# Autodesk Inventor assembly: PI-101
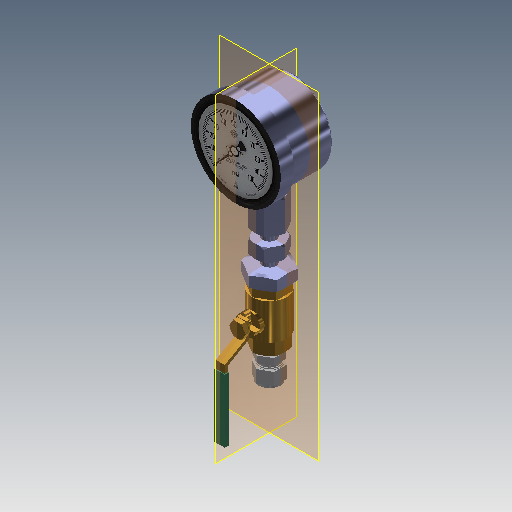
[picture p0: Inventor's stored thumbnail of the model, 512x512]
Saved by Autodesk Inventor 2020 (Build 240152000, 152)
## iProperties
Created: 2009-08-11
Part Number: PI-101
Document SubType Name: Assembly
Designer: Demir Ali
Mass: 1096.47 g
Surface Area: 738.205 cm^2
Volume: 566.838 cm^3
Density: 1.93437 g/cm^3
Description: Pressure Gauge
Stock Number: NA
Author: Demir Ali
Title: Purchased Part
Revision Number: A
## Documents named in this file (4)
- C:\Users\hallc\Desktop\Process Equipment\Workspace\Supplier Content\Pressure Gauge\PI-101.iam
- C:\Users\hallc\Desktop\Process Equipment\Libraries\Content Center Files\en-US\Parker A(28)\Parker A-Lok Male Taper Thread - Metric Tube M15 x 1_2.ipt
- C:\Users\hallc\Desktop\Process Equipment\Libraries\Content Center Files\en-US\Pressure Gauge-PN16 BSPT Thread\Pressure Gauge - 0.75 in BSP.ipt
- C:\Users\hallc\Desktop\Process Equipment\Libraries\Content Center Files\en-US\Parker XV500P\Parker Female-Female Pipe Ends XV500P XV500P-12.ipt
## Components (3 placed, 3 different names)
1. Parker A-Lok Male Taper Thread - Metric Tube M15 x 1/2:1 — Insert:2
2. Pressure Gauge-PN16 BSPT Thread 19.05:1 — Insert:1, Angle:1
3. Parker Female-Female Pipe Ends XV500P XV500P-12:1 — Insert:1, Insert:2, Angle:1, Flush:1
## Relationships (4: Insert 2, Angle 1, Flush 1)
- Insert:1: Pressure Gauge-PN16 BSPT Thread 19.05:1 ↔ Parker Female-Female Pipe Ends XV500P XV500P-12:1
- Insert:2: Parker A-Lok Male Taper Thread - Metric Tube M15 x 1/2:1 ↔ Parker Female-Female Pipe Ends XV500P XV500P-12:1
- Angle:1 (180 deg): Pressure Gauge-PN16 BSPT Thread 19.05:1 ↔ Parker Female-Female Pipe Ends XV500P XV500P-12:1
- Flush:1: Parker Female-Female Pipe Ends XV500P XV500P-12:1
